# Autodesk Inventor assembly: halfcut-48t-gear
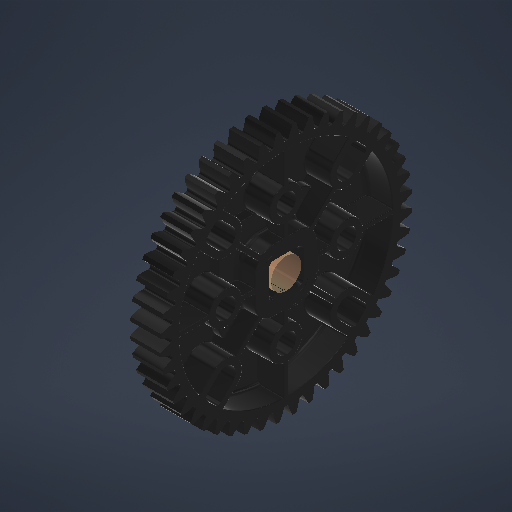
[picture p0: Inventor's stored thumbnail of the model, 512x512]
Saved by Autodesk Inventor 2025.1 (Build 291241000, 241)
## iProperties
Created: 2025-07-20
Part Number: halfcut-48t-gear
Document SubType Name: Assembly
Designer: Exortions
Author: Exortions
## Documents named in this file (3)
- D:\Robotics\jank-2025-3284B\cad3284b-2025\highlander\parts\halfcut-48t-gear.iam
- D:\Robotics\jank-2025-3284B\cad3284b-2025\VEX-CAD-Inventor-1.4.2\Motion\Gears\HS Gear\HS 48T Gear, No Insert.iam
- D:\Robotics\jank-2025-3284B\cad3284b-2025\VEX-CAD-Inventor-1.4.2\Motion\Gears\HS Gear.iam
## Components (1 placed, 1 different names)
1. HS 48T Gear, No Insert:1 [sub-assembly] — Flush:1
## Relationships (1: Flush 1)
- Flush:1: HS 48T Gear, No Insert:1
